# Autodesk Inventor assembly: objectRetrieval
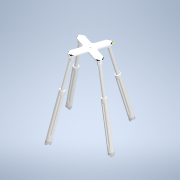
[picture p0: Inventor's stored thumbnail of the model, 180x180]
Saved by Autodesk Inventor 2022 (Build 260153000, 153)
## iProperties
Created: 2022-04-28
Part Number: objectRetrieval
Document SubType Name: Assembly
Designer: Dahway
Author: Dahway
## Documents named in this file (5)
- C:\Users\Dahway\Documents\GitHub\GMU-RobotX-Mechanical\Object Retrieval\V3\objectRetrieval.iam
- C:\Users\Dahway\Documents\GitHub\GMU-RobotX-Mechanical\Object Retrieval\V3\armLower.ipt
- C:\Users\Dahway\Documents\GitHub\GMU-RobotX-Mechanical\Object Retrieval\V3\armPlug.ipt
- C:\Users\Dahway\Documents\GitHub\GMU-RobotX-Mechanical\Object Retrieval\V3\armUpper.ipt
- C:\Users\Dahway\Documents\GitHub\GMU-RobotX-Mechanical\Object Retrieval\V3\equipPlate.ipt
## Components (13 placed, 4 different names)
1. equipPlate:1 — Mate:7, Mate:8, Mate:9, Mate:10
2. armLower:1 — Mate:1, Mate:2, Mate:6, Mate:8, Mate:9, Mate:10
3. armPlug:1 — Mate:3, Mate:4, Mate:5
4. armUpper:1 — Mate:1, Mate:2, Mate:3, Mate:4, Mate:5, Mate:6
5. armLower:2
6. armPlug:2
7. armUpper:2
8. armLower:3
9. armPlug:3
10. armUpper:3
11. armLower:4
12. armPlug:4
13. armUpper:4
## Component patterns: (4 elements, first: armLower:1 + armPlug:1 + armUpper:1)
## Relationships (10: Mate 10)
- Mate:1: armLower:1 ↔ armUpper:1
- Mate:2: armLower:1 ↔ armUpper:1
- Mate:3: armPlug:1 ↔ armUpper:1
- Mate:4: armPlug:1 ↔ armUpper:1
- Mate:5: armPlug:1 ↔ armUpper:1
- Mate:6: armLower:1 ↔ armUpper:1
- Mate:7: equipPlate:1
- Mate:8 (0.508 mm): equipPlate:1 ↔ armLower:1
- Mate:9 (2.54 mm): equipPlate:1 ↔ armLower:1
- Mate:10: equipPlate:1 ↔ armLower:1
